# Autodesk Inventor assembly: FRAME
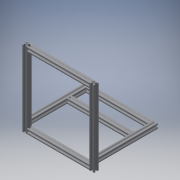
[picture p0: Inventor's stored thumbnail of the model, 180x180]
Saved by Autodesk Inventor 2018 (Build 220112000, 112)
## iProperties
Created: 2018-10-12
Part Number: FRAME
Document SubType Name: Assembly
Designer: mam373
Author: mam373
## Documents named in this file (4)
- C:\Users\mam37\OneDrive\Documents\Fall 2018\TECH 4398\FRAME (1).iam
- C:\Users\mam37\OneDrive\Documents\Fall 2018\TECH 4398\T-SLOT A.ipt
- C:\Users\mam37\OneDrive\Documents\Fall 2018\TECH 4398\T-SLOT B.ipt
- C:\Users\mam37\OneDrive\Documents\Fall 2018\TECH 4398\T-SLOT C.ipt
## Components (8 placed, 3 different names)
1. T-SLOT A:1 — Mate:1, Flush:1, Flush:2, Mate:2, Flush:3, Flush:4, Mate:4, Flush:7, Flush:12
2. T-SLOT A:2 — Mate:3, Flush:5, Flush:6, Mate:5, Flush:8, Flush:13
3. T-SLOT B:1 — Mate:1, Flush:1, Flush:2
4. T-SLOT B:2 — Mate:2, Flush:3, Flush:4, Mate:3, Flush:5, Flush:6
5. T-SLOT C:1 — Mate:4, Flush:7, Mate:6, Flush:9, Flush:10, Mate:7, Flush:11, Flush:12
6. T-SLOT C:2 — Mate:5, Flush:8, Flush:13
7. T-SLOT B:3 — Mate:7, Flush:11, Mate:8
8. T-SLOT B:4 — Mate:6, Flush:9, Flush:10, Mate:8
## Relationships (21: Flush 13, Mate 8)
- Mate:1: T-SLOT A:1 ↔ T-SLOT B:1
- Flush:1: T-SLOT A:1 ↔ T-SLOT B:1
- Flush:2: T-SLOT A:1 ↔ T-SLOT B:1
- Mate:2: T-SLOT A:1 ↔ T-SLOT B:2
- Flush:3: T-SLOT A:1 ↔ T-SLOT B:2
- Flush:4: T-SLOT A:1 ↔ T-SLOT B:2
- Mate:3: T-SLOT A:2 ↔ T-SLOT B:2
- Flush:5: T-SLOT A:2 ↔ T-SLOT B:2
- Flush:6: T-SLOT A:2 ↔ T-SLOT B:2
- Mate:4: T-SLOT A:1 ↔ T-SLOT C:1
- Flush:7: T-SLOT A:1 ↔ T-SLOT C:1
- Mate:5: T-SLOT A:2 ↔ T-SLOT C:2
- Flush:8: T-SLOT A:2 ↔ T-SLOT C:2
- Mate:6: T-SLOT C:1 ↔ T-SLOT B:4
- Flush:9: T-SLOT C:1 ↔ T-SLOT B:4
- Flush:10: T-SLOT C:1 ↔ T-SLOT B:4
- Mate:7: T-SLOT C:1 ↔ T-SLOT B:3
- Flush:11: T-SLOT C:1 ↔ T-SLOT B:3
- Flush:12 (-25.4 mm): T-SLOT A:1 ↔ T-SLOT C:1
- Flush:13 (-25.4 mm): T-SLOT A:2 ↔ T-SLOT C:2
- Mate:8 (57.15 mm): T-SLOT B:3 ↔ T-SLOT B:4
